# Autodesk Inventor assembly: Fuehrungsrollen_Assembly
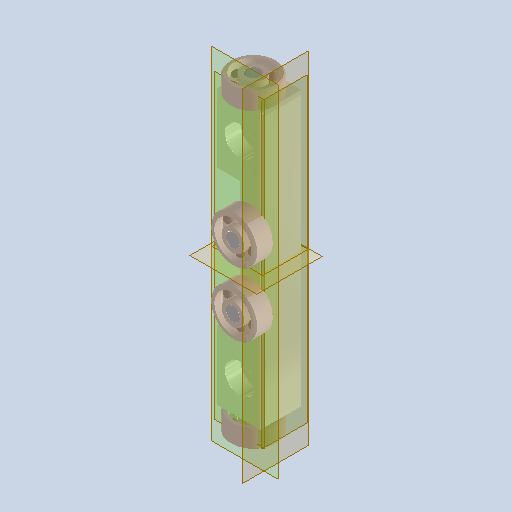
[picture p0: Inventor's stored thumbnail of the model, 512x512]
Saved by Autodesk Inventor 2024 (Build 280153000, 153)
## iProperties
Created: 2022-08-16
Part Number: Fuehrungsrollen_Assembly
Document SubType Name: Assembly
Designer: alexw
Mass: 7.20177 g
Surface Area: 50.3407 cm^2
Volume: 4.5105 cm^3
Author: alexw
## Documents named in this file (4)
- C:\Users\AEWALDER\Documents\Inventor\03_CurrentProjects\MasterThesis\PSM_V1_Rillenkugellager\Ueberarbeiteter DaVincikopf\Fuehrungsrollen_Assembly.iam
- C:\Users\AEWALDER\Documents\Inventor\03_CurrentProjects\MasterThesis\PSM_V1_Rillenkugellager\Ueberarbeiteter DaVincikopf\Fuehrungslagerhalter_v2.ipt
- C:\Users\AEWALDER\Documents\Inventor\03_CurrentProjects\MasterThesis\PSM_V1_Rillenkugellager\Ueberarbeiteter DaVincikopf\Lager.iam
- C:\Users\AEWALDER\Documents\Inventor\03_CurrentProjects\MasterThesis\PSM_V1_Rillenkugellager\Ueberarbeiteter DaVincikopf\3mmSchaft_10mm.ipt
## Components (9 placed, 3 different names)
1. Fuehrungslagerhalter_v2:1 — Passend:2, Passend:3, Passend:4, Passend:5, Passend:6, Passend:7, Passend:8, Fluchtend:1, Fluchtend:2, Passend:9
2. Lager:1 [sub-assembly]
3. Lager:2 [sub-assembly]
4. Lager:3 [sub-assembly]
5. Lager:4 [sub-assembly]
6. 3mmSchaft_10mm:1 — Passend:2
7. 3mmSchaft_10mm:2 — Passend:3, Passend:7
8. 3mmSchaft_10mm:3 — Passend:4, Passend:6
9. 3mmSchaft_10mm:4 — Passend:5, Passend:8
## Relationships (15: Mate 9, RevoluteJoint 4, Flush 2)
- [RevoluteJoint]: Fuehrungslagerhalter_v2:1 ↔ Lager:4
- [RevoluteJoint]: Fuehrungslagerhalter_v2:1 ↔ Lager:3
- [RevoluteJoint]: Fuehrungslagerhalter_v2:1 ↔ Lager:1
- [RevoluteJoint]: Fuehrungslagerhalter_v2:1 ↔ Lager:2
- [Mate]: Fuehrungslagerhalter_v2:1 ↔ 3mmSchaft_10mm:1
- Passend:2 [Mate]: Fuehrungslagerhalter_v2:1 ↔ 3mmSchaft_10mm:1
- Passend:3 [Mate]: Fuehrungslagerhalter_v2:1 ↔ 3mmSchaft_10mm:2
- Passend:4 [Mate]: Fuehrungslagerhalter_v2:1 ↔ 3mmSchaft_10mm:3
- Passend:5 [Mate]: Fuehrungslagerhalter_v2:1 ↔ 3mmSchaft_10mm:4
- Passend:6 [Mate]: Fuehrungslagerhalter_v2:1 ↔ 3mmSchaft_10mm:3
- Passend:7 [Mate]: Fuehrungslagerhalter_v2:1 ↔ 3mmSchaft_10mm:2
- Passend:8 [Mate]: Fuehrungslagerhalter_v2:1 ↔ 3mmSchaft_10mm:4
- Fluchtend:1 [Flush]: Fuehrungslagerhalter_v2:1
- Fluchtend:2 [Flush]: Fuehrungslagerhalter_v2:1
- Passend:9 [Mate]: Fuehrungslagerhalter_v2:1
